# Autodesk Inventor assembly: 08-3
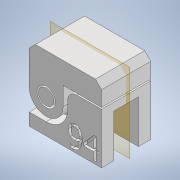
[picture p0: Inventor's stored thumbnail of the model, 180x180]
Saved by Autodesk Inventor 2022 (Build 260153000, 153)
## iProperties
Created: 2021-09-11
Part Number: 08-3
Document SubType Name: Assembly
Designer: 서울공업고등학교
Author: 서울공업고등학교
## Documents named in this file (3)
- C:\Users\서울공업고등학교\Documents\_9_11\모의고사8\08-3.iam
- C:\Users\서울공업고등학교\Documents\_9_11\모의고사8\1번부품.ipt
- C:\Users\서울공업고등학교\Documents\_9_11\모의고사8\2번부품.ipt
## Components (2 placed, 2 different names)
1. 1번부품:1 — 플러쉬:1, 메이트:1
2. 2번부품:1 — 플러쉬:1, 메이트:1
## Relationships (2: Flush 1, Mate 1)
- 플러쉬:1 [Flush]: 1번부품:1 ↔ 2번부품:1
- 메이트:1 [Mate]: 1번부품:1 ↔ 2번부품:1
